# Autodesk Inventor assembly: Gear Reduction Unit
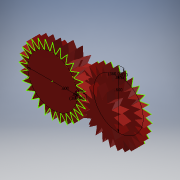
[picture p0: Inventor's stored thumbnail of the model, 180x180]
Saved by Autodesk Inventor 2017 (Build 210142000, 142)
## iProperties
Created: 2018-09-18
Part Number: Gear Reduction Unit
Document SubType Name: Assembly
Designer: User
Author: User
## Documents named in this file (4)
- E:\Gear Reduction Unit.iam
- E:\Big Gear Phone Case Mech.ipt
- E:\Small Gear Phone Case Mech.ipt
- E:\Gear Set With Spacer.iam
## Components (4 placed, 3 different names)
1. Big Gear Phone Case Mech:1 — Insert:1
2. Small Gear Phone Case Mech:1 — Insert:1, Flush:1, Mate:1, Insert:2
3. Gear Set With Spacer:1 [sub-assembly] — Flush:1, Mate:1
4. Big Gear Phone Case Mech:2 — Insert:2
## Relationships (4: Insert 2, Flush 1, Mate 1)
- Insert:1: Big Gear Phone Case Mech:1 ↔ Small Gear Phone Case Mech:1
- Flush:1: Small Gear Phone Case Mech:1 ↔ Gear Set With Spacer:1
- Mate:1: Small Gear Phone Case Mech:1 ↔ Gear Set With Spacer:1
- Insert:2: Small Gear Phone Case Mech:1 ↔ Big Gear Phone Case Mech:2
